# Autodesk Inventor assembly: Chassis
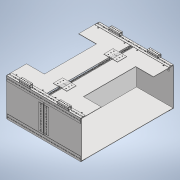
[picture p0: Inventor's stored thumbnail of the model, 180x180]
Saved by Autodesk Inventor 2020 (Build 240168000, 168)
## iProperties
Created: 2021-11-11
Part Number: Chassis
Document SubType Name: Assembly
Designer: 17185
Author: 17185
## Documents named in this file (3)
- C:\Users\17185\Desktop\chassis draft\Chassis Frame\Chassis.iam
- C:\Users\17185\Desktop\chassis draft\Chassis Frame\ChassisFrame.iam
- C:\Users\17185\Desktop\chassis draft\DriveHousing\DriveHousing.iam
## Components (3 placed, 2 different names)
1. ChassisFrame:1 [sub-assembly] — Mate:1, Mate:2, Mate:3, Mate:4, Mate:5, Mate:6
2. DriveHousing:1 [sub-assembly] — Mate:1, Mate:2, Mate:3
3. DriveHousing:2 [sub-assembly] — Mate:4, Mate:5, Mate:6
## Relationships (6: Mate 6)
- Mate:1: ChassisFrame:1 ↔ DriveHousing:1
- Mate:2: ChassisFrame:1 ↔ DriveHousing:1
- Mate:3: ChassisFrame:1 ↔ DriveHousing:1
- Mate:4: ChassisFrame:1 ↔ DriveHousing:2
- Mate:5: ChassisFrame:1 ↔ DriveHousing:2
- Mate:6: ChassisFrame:1 ↔ DriveHousing:2
